# Autodesk Inventor assembly: Link_4
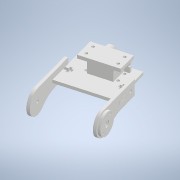
[picture p0: Inventor's stored thumbnail of the model, 180x180]
Saved by Autodesk Inventor 2022 (Build 260153000, 153)
## iProperties
Created: 2021-09-23
Part Number: Link_4
Document SubType Name: Assembly
Designer: Administrador
Author: Administrador
## Documents named in this file (7)
- C:\Users\Administrador\Desktop\Octavo Semestre\Robótica Industrial\Robot\Links\Link_4.iam
- C:\Users\Administrador\Desktop\Octavo Semestre\Robótica Industrial\Robot\Cuerpo\PartesCuerpo\Brazo3Izquierda.ipt
- C:\Users\Administrador\Desktop\Octavo Semestre\Robótica Industrial\Robot\Cuerpo\PartesCuerpo\Brazo3.ipt
- C:\Users\Administrador\Desktop\Octavo Semestre\Robótica Industrial\Robot\Cuerpo\PartesCuerpo\Circulo_Inferior.ipt
- C:\Users\Administrador\Desktop\Octavo Semestre\Robótica Industrial\Robot\Cuerpo\PartesCuerpo\Muñeca1.ipt
- C:\Users\Administrador\Desktop\Octavo Semestre\Robótica Industrial\Robot\Cuerpo\PartesCuerpo\Muñeca2.ipt
- C:\Users\Administrador\Desktop\Octavo Semestre\Robótica Industrial\Robot\Cuerpo\PartesCuerpo\Microservo Mg90.ipt
## Components (6 placed, 6 different names)
1. Brazo3Izquierda:1
2. Brazo3:1
3. Circulo_Inferior:1
4. Muñeca1:1
5. Muñeca2:1
6. Microservo Mg90:1
## Relationships (11: Mate 8, Flush 3)
- [Mate]: Brazo3:1 ↔ Circulo_Inferior:1
- [Mate]: Brazo3:1 ↔ Circulo_Inferior:1
- [Mate]: Brazo3Izquierda:1 ↔ Brazo3:1
- [Flush]: Brazo3:1 ↔ Muñeca1:1
- [Mate]: Brazo3:1 ↔ Muñeca1:1
- [Mate]: Brazo3:1 ↔ Muñeca1:1
- [Mate]: Muñeca1:1 ↔ Microservo Mg90:1
- [Mate] (13 mm): Brazo3:1 ↔ Microservo Mg90:1
- [Flush]: Muñeca1:1 ↔ Microservo Mg90:1
- [Mate]: Muñeca2:1 ↔ Microservo Mg90:1
- [Flush] (4.3 mm): Muñeca2:1 ↔ Microservo Mg90:1
